# Autodesk Inventor assembly: electrical board back
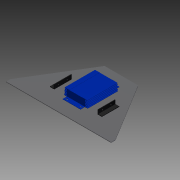
[picture p0: Inventor's stored thumbnail of the model, 180x180]
Saved by Autodesk Inventor 2012 (Build 160160000, 160)
## iProperties
Created: 2011-10-06
Part Number: electrical board back
Document SubType Name: Assembly
Designer: Antonella
Author: Antonella
## Documents named in this file (4)
- C:\Users\Antonella\Documents\GCC Robotics 2012 - Mechanical\Robot 2.0\Electrical\Back Electrical Board\Bottom\Electrical Board - back bottom.iam
- C:\Users\Antonella\Documents\GCC Robotics 2012 - Mechanical\Robot 2.0\Electrical\Back Electrical Board\Bottom\Electrical Board - back bottom.ipt
- C:\Users\Antonella\Documents\GCC Robotics 2012 - Mechanical\Robot 2.0\Electrical\Roboteq_HDC2450\Roboteq_HDC2450.ipt
- C:\Users\Antonella\Documents\GCC Robotics 2012 - Mechanical\Robot 2.0\Electrical\Back Electrical Board\top board mount bracket.ipt
## Components (4 placed, 3 different names)
1. Electrical Board - back bottom:1 — Mate:1, Flush:1, Flush:2, Mate:2, Flush:3, Mate:3, Mate:5, Mate:6
2. Roboteq_HDC2450:1 — Mate:1, Flush:1, Flush:2
3. top board mount bracket:1 — Mate:3, Mate:4, Mate:6
4. top board mount bracket:2 — Mate:2, Flush:3, Mate:4, Mate:5
## Relationships (9: Mate 6, Flush 3)
- Mate:1: Electrical Board - back bottom:1 ↔ Roboteq_HDC2450:1
- Flush:1 (63.5 mm): Electrical Board - back bottom:1 ↔ Roboteq_HDC2450:1
- Flush:2: Electrical Board - back bottom:1 ↔ Roboteq_HDC2450:1
- Mate:2: Electrical Board - back bottom:1 ↔ top board mount bracket:2
- Flush:3 (101.6 mm): Electrical Board - back bottom:1 ↔ top board mount bracket:2
- Mate:3: Electrical Board - back bottom:1 ↔ top board mount bracket:1
- Mate:4: top board mount bracket:1 ↔ top board mount bracket:2
- Mate:5 (-127 mm): Electrical Board - back bottom:1 ↔ top board mount bracket:2
- Mate:6 (127 mm): Electrical Board - back bottom:1 ↔ top board mount bracket:1
